# Autodesk Inventor assembly: CCM_Unit
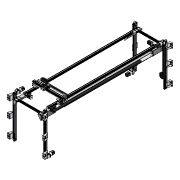
[picture p0: Inventor's stored thumbnail of the model, 180x180]
Saved by Autodesk Inventor 2020 (Build 240168000, 168)
## iProperties
Created: 2021-02-24
Part Number: CCM_Unit
Document SubType Name: Assembly
Designer: magnarecta
Author: magnarecta
## Documents named in this file (19)
- D:\Documents\GitHub\Eto_Project\Hardware\Asem\CCM_Unit.iam
- D:\Documents\GitHub\Eto_Project\Hardware\Parts\CCM\CCM motion linear guide rail\CCM_UNIT\CCM_Unit_C.iam
- D:\Documents\GitHub\Eto_Project\Hardware\Parts\CCM\CCM motion linear guide rail\CCM_UNIT\CCM_Unit_B.iam
- D:\Documents\GitHub\Eto_Project\Hardware\Parts\Stepper_Motor\NEMA23 Stepper.ipt
- D:\Documents\GitHub\Eto_Project\Hardware\Parts\CCM\CCM motion linear guide rail\CCM_UNIT\CCM_Unit_D.iam
- D:\Documents\GitHub\Eto_Project\Hardware\Parts\Meviy\New_Meviy\CCM_Mount_B.ipt
- D:\Documents\GitHub\Eto_Project\Hardware\Parts\Meviy\New_Meviy\CCM_Mount_C.ipt
- D:\Documents\GitHub\Eto_Project\Hardware\Parts\Meviy\New_Meviy\CCM_Mount_D.ipt
- D:\Documents\GitHub\Eto_Project\Hardware\Parts\Meviy\New_Meviy\CCM_Mount_E.ipt
- D:\Documents\GitHub\Eto_Project\Hardware\Parts\Meviy\New_Meviy\CCM_Mount_F.ipt
- D:\Documents\GitHub\Eto_Project\Hardware\Parts\Meviy\New_Meviy\CCM_Mount_G.ipt
- D:\Documents\GitHub\Eto_Project\Hardware\Parts\MISUMI\SLHSSW10_Autodesk_Inventor_2020_20211206\AIS2020\SLHSSW10.iam
- D:\Documents\GitHub\Eto_Project\Hardware\Parts\MISUMI\PSSFGW10-582-M6-N6_Autodesk_Inventor_2020_20211206\PSSFGW10-582-M6-N6.ipt
- D:\Documents\GitHub\Eto_Project\Hardware\Parts\Cable chain\J15BF.1.30_Xaxis.ipt
- D:\Documents\GitHub\Eto_Project\Hardware\Parts\Cable chain\J15BF.1.30_Yaxis.ipt
- D:\Documents\GitHub\Eto_Project\Hardware\Parts\Meviy\New_Meviy\DragChain_Guide_A.ipt
- D:\Documents\GitHub\Eto_Project\Hardware\Parts\Cable chain\J15BF.1.30_Zaxis.ipt
- D:\Documents\GitHub\Eto_Project\Hardware\Parts\Meviy\New_Meviy\DragChain_Guide_B.ipt
- D:\Documents\GitHub\Eto_Project\Hardware\Parts\MISUMI\HFSB6-3030-586-HPW_Autodesk_Inventor_2020_20211208\HFSB6-3030-586-HPW.ipt
## Components (40 placed, 18 different names)
1. CCM_Unit_B:1 [sub-assembly] — 挿入:9, 角度:3, メイト:4, メイト:5, 角度:8, メイト:14, メイト:16, フラッシュ:21, 挿入:37, 挿入:38, メイト:36, フラッシュ:23, メイト:41
2. NEMA23 Stepper:1 — 挿入:12, 角度:5
3. NEMA23 Stepper:2 — 挿入:9, 角度:3
4. CCM_Unit_C:2 [sub-assembly] — メイト:8, メイト:9, フラッシュ:13, フラッシュ:14, フラッシュ:15, フラッシュ:18, 挿入:19, 挿入:20
5. CCM_Unit_D:1 [sub-assembly] — 挿入:12, 角度:5, フラッシュ:20, メイト:35, メイト:36, フラッシュ:26
6. CCM_Unit_B:2 [sub-assembly] — メイト:4, メイト:5, 角度:7, フラッシュ:20, 挿入:35, 挿入:36, フラッシュ:21, フラッシュ:22
7. NEMA23 Stepper:4
8. CCM_Unit_C:3 [sub-assembly] — 角度:7, メイト:8, メイト:9, フラッシュ:16, メイト:12, フラッシュ:17, 挿入:17, 挿入:18
9. CCM_Unit_C:4 [sub-assembly] — フラッシュ:16, メイト:12, メイト:13, メイト:14, フラッシュ:17, フラッシュ:19, 挿入:33, 挿入:34
10. CCM_Unit_C:5 [sub-assembly] — フラッシュ:13, 角度:8, フラッシュ:14, フラッシュ:15, メイト:13, フラッシュ:18, フラッシュ:19, メイト:15, 挿入:15, 挿入:16, メイト:45, 挿入:41, 挿入:42
11. CCM_Mount_B:2 — メイト:15, メイト:16, メイト:17, メイト:18, メイト:19, メイト:20, メイト:21, メイト:22, メイト:23, メイト:24, 挿入:15, 挿入:16, メイト:25, フラッシュ:23, メイト:44, 角度:11
12. CCM_Mount_C:1 — メイト:17, メイト:18, メイト:19
13. CCM_Mount_D:1 — メイト:23, メイト:24, メイト:25
14. CCM_Mount_D:2 — メイト:20, メイト:21, メイト:22, メイト:43, 角度:10
15. CCM_Mount_B:3 — 挿入:17, 挿入:18, 挿入:43
16. CCM_Mount_C:2
17. CCM_Mount_D:3
18. CCM_Mount_D:4
19. CCM_Mount_E:1 — 挿入:19, 挿入:20, 挿入:21, 挿入:22, 挿入:23, 挿入:24, 挿入:25, 挿入:26, フラッシュ:22, 挿入:44
20. CCM_Mount_C:3 — 挿入:21, 挿入:22
21. CCM_Mount_D:5 — 挿入:23, 挿入:24
22. CCM_Mount_C:4 — 挿入:25, 挿入:26
23. CCM_Mount_E:2 — 挿入:33, 挿入:34, フラッシュ:30, 角度:12
24. CCM_Mount_C:5
25. CCM_Mount_D:6
26. CCM_Mount_C:6
27. CCM_Mount_F:1 — 挿入:35, 挿入:36, メイト:35, メイト:38, フラッシュ:28
28. CCM_Mount_G:1 — 挿入:37, 挿入:38, メイト:37, 挿入:39, 挿入:40, フラッシュ:27, メイト:39, メイト:40, 角度:9, フラッシュ:29
29. SLHSSW10:1 [sub-assembly] — メイト:37, フラッシュ:24, フラッシュ:25
30. SLHSSW10:2 [sub-assembly] — メイト:38, フラッシュ:24, フラッシュ:25, フラッシュ:26
31. PSSFGW10-582-M6-N6:1 — 挿入:39
32. PSSFGW10-582-M6-N6:2 — 挿入:40
33. J15BF.1.30_Xaxis:2 — フラッシュ:27, フラッシュ:28, メイト:39
34. J15BF.1.30_Yaxis:1 — メイト:40, 角度:9, フラッシュ:29
35. DragChain_Guide_A:1 — メイト:41, フラッシュ:30, フラッシュ:31, フラッシュ:32, メイト:42
36. DragChain_Guide_A:2 — フラッシュ:31, フラッシュ:32, メイト:42, メイト:43
37. J15BF.1.30_Zaxis:1 — メイト:44, 角度:10, メイト:45, フラッシュ:33
38. DragChain_Guide_B:1 — 挿入:41, 挿入:42, フラッシュ:33
39. HFSB6-3030-586-HPW:1 — 挿入:43, 角度:12
40. HFSB6-3030-586-HPW:2 — 挿入:44, 角度:11
## Relationships (103: Mate 40, Insert 33, Flush 21, Angle 9)
- 挿入:9 [Insert] (2 mm): CCM_Unit_B:1 ↔ NEMA23 Stepper:2
- 角度:3 [Angle] (0 deg): CCM_Unit_B:1 ↔ NEMA23 Stepper:2
- 挿入:12 [Insert] (5 mm): NEMA23 Stepper:1 ↔ CCM_Unit_D:1
- 角度:5 [Angle] (0 deg): NEMA23 Stepper:1 ↔ CCM_Unit_D:1
- [Insert] (2 mm): CCM_Unit_B:2 ↔ NEMA23 Stepper:4
- [Angle] (0 deg): CCM_Unit_B:2 ↔ NEMA23 Stepper:4
- メイト:4 [Mate]: CCM_Unit_B:1 ↔ CCM_Unit_B:2
- メイト:5 [Mate]: CCM_Unit_B:1 ↔ CCM_Unit_B:2
- 角度:7 [Angle] (180 deg): CCM_Unit_B:2 ↔ CCM_Unit_C:3
- メイト:8 [Mate]: CCM_Unit_C:2 ↔ CCM_Unit_C:3
- メイト:9 [Mate]: CCM_Unit_C:2 ↔ CCM_Unit_C:3
- [Mate]: CCM_Unit_C:4 ↔ CCM_Unit_C:5
- [Mate]: CCM_Unit_C:4 ↔ CCM_Unit_C:5
- フラッシュ:13 [Flush]: CCM_Unit_C:2 ↔ CCM_Unit_C:5
- 角度:8 [Angle] (180 deg): CCM_Unit_B:1 ↔ CCM_Unit_C:5
- フラッシュ:14 [Flush]: CCM_Unit_C:2 ↔ CCM_Unit_C:5
- フラッシュ:15 [Flush]: CCM_Unit_C:2 ↔ CCM_Unit_C:5
- フラッシュ:16 [Flush]: CCM_Unit_C:3 ↔ CCM_Unit_C:4
- メイト:12 [Mate] (686 mm): CCM_Unit_C:3 ↔ CCM_Unit_C:4
- メイト:13 [Mate] (2488 mm): CCM_Unit_C:4 ↔ CCM_Unit_C:5
- メイト:14 [Mate] (136.5 mm): CCM_Unit_B:1 ↔ CCM_Unit_C:4
- フラッシュ:17 [Flush]: CCM_Unit_C:3 ↔ CCM_Unit_C:4
- フラッシュ:18 [Flush]: CCM_Unit_C:2 ↔ CCM_Unit_C:5
- フラッシュ:19 [Flush]: CCM_Unit_C:4 ↔ CCM_Unit_C:5
- メイト:15 [Mate]: CCM_Unit_C:5 ↔ CCM_Mount_B:2
- メイト:16 [Mate]: CCM_Unit_B:1 ↔ CCM_Mount_B:2
- メイト:17 [Mate]: CCM_Mount_B:2 ↔ CCM_Mount_C:1
- メイト:18 [Mate]: CCM_Mount_B:2 ↔ CCM_Mount_C:1
- メイト:19 [Mate]: CCM_Mount_B:2 ↔ CCM_Mount_C:1
- メイト:20 [Mate]: CCM_Mount_B:2 ↔ CCM_Mount_D:2
- メイト:21 [Mate]: CCM_Mount_B:2 ↔ CCM_Mount_D:2
- メイト:22 [Mate]: CCM_Mount_B:2 ↔ CCM_Mount_D:2
- メイト:23 [Mate]: CCM_Mount_B:2 ↔ CCM_Mount_D:1
- メイト:24 [Mate]: CCM_Mount_B:2 ↔ CCM_Mount_D:1
- 挿入:15 [Insert]: CCM_Unit_C:5 ↔ CCM_Mount_B:2
- 挿入:16 [Insert]: CCM_Unit_C:5 ↔ CCM_Mount_B:2
- メイト:25 [Mate]: CCM_Mount_B:2 ↔ CCM_Mount_D:1
- [Mate]: CCM_Mount_B:3 ↔ CCM_Mount_C:2
- [Mate]: CCM_Mount_B:3 ↔ CCM_Mount_C:2
- [Mate]: CCM_Mount_B:3 ↔ CCM_Mount_C:2
- [Mate]: CCM_Mount_B:3 ↔ CCM_Mount_D:4
- [Mate]: CCM_Mount_B:3 ↔ CCM_Mount_D:4
- [Mate]: CCM_Mount_B:3 ↔ CCM_Mount_D:4
- [Mate]: CCM_Mount_B:3 ↔ CCM_Mount_D:3
- [Mate]: CCM_Mount_B:3 ↔ CCM_Mount_D:3
- [Mate]: CCM_Mount_B:3 ↔ CCM_Mount_D:3
- 挿入:17 [Insert]: CCM_Unit_C:3 ↔ CCM_Mount_B:3
- 挿入:18 [Insert]: CCM_Unit_C:3 ↔ CCM_Mount_B:3
- 挿入:19 [Insert]: CCM_Unit_C:2 ↔ CCM_Mount_E:1
- 挿入:20 [Insert]: CCM_Unit_C:2 ↔ CCM_Mount_E:1
- 挿入:21 [Insert]: CCM_Mount_E:1 ↔ CCM_Mount_C:3
- 挿入:22 [Insert]: CCM_Mount_E:1 ↔ CCM_Mount_C:3
- 挿入:23 [Insert]: CCM_Mount_E:1 ↔ CCM_Mount_D:5
- 挿入:24 [Insert]: CCM_Mount_E:1 ↔ CCM_Mount_D:5
- 挿入:25 [Insert]: CCM_Mount_E:1 ↔ CCM_Mount_C:4
- 挿入:26 [Insert]: CCM_Mount_E:1 ↔ CCM_Mount_C:4
- [Insert]: CCM_Mount_E:2 ↔ CCM_Mount_C:5
- [Insert]: CCM_Mount_E:2 ↔ CCM_Mount_C:5
- [Insert]: CCM_Mount_E:2 ↔ CCM_Mount_D:6
- [Insert]: CCM_Mount_E:2 ↔ CCM_Mount_D:6
- [Insert]: CCM_Mount_E:2 ↔ CCM_Mount_C:6
- [Insert]: CCM_Mount_E:2 ↔ CCM_Mount_C:6
- 挿入:33 [Insert]: CCM_Unit_C:4 ↔ CCM_Mount_E:2
- 挿入:34 [Insert]: CCM_Unit_C:4 ↔ CCM_Mount_E:2
- フラッシュ:20 [Flush] (-27 mm): CCM_Unit_D:1 ↔ CCM_Unit_B:2
- 挿入:35 [Insert]: CCM_Unit_B:2 ↔ CCM_Mount_F:1
- 挿入:36 [Insert]: CCM_Unit_B:2 ↔ CCM_Mount_F:1
- メイト:35 [Mate]: CCM_Unit_D:1 ↔ CCM_Mount_F:1
- フラッシュ:21 [Flush]: CCM_Unit_B:1 ↔ CCM_Unit_B:2
- 挿入:37 [Insert]: CCM_Unit_B:1 ↔ CCM_Mount_G:1
- 挿入:38 [Insert]: CCM_Unit_B:1 ↔ CCM_Mount_G:1
- メイト:36 [Mate] (20 mm): CCM_Unit_B:1 ↔ CCM_Unit_D:1
- フラッシュ:22 [Flush]: CCM_Unit_B:2 ↔ CCM_Mount_E:1
- フラッシュ:23 [Flush]: CCM_Unit_B:1 ↔ CCM_Mount_B:2
- メイト:37 [Mate]: CCM_Mount_G:1 ↔ SLHSSW10:1
- メイト:38 [Mate]: CCM_Mount_F:1 ↔ SLHSSW10:2
- フラッシュ:24 [Flush]: SLHSSW10:1 ↔ SLHSSW10:2
- フラッシュ:25 [Flush]: SLHSSW10:1 ↔ SLHSSW10:2
- フラッシュ:26 [Flush] (5 mm): CCM_Unit_D:1 ↔ SLHSSW10:2
- 挿入:39 [Insert]: CCM_Mount_G:1 ↔ PSSFGW10-582-M6-N6:1
- 挿入:40 [Insert]: CCM_Mount_G:1 ↔ PSSFGW10-582-M6-N6:2
- フラッシュ:27 [Flush]: CCM_Mount_G:1 ↔ J15BF.1.30_Xaxis:2
- フラッシュ:28 [Flush]: CCM_Mount_F:1 ↔ J15BF.1.30_Xaxis:2
- メイト:39 [Mate]: CCM_Mount_G:1 ↔ J15BF.1.30_Xaxis:2
- メイト:40 [Mate]: CCM_Mount_G:1 ↔ J15BF.1.30_Yaxis:1
- 角度:9 [Angle] (0 deg): CCM_Mount_G:1 ↔ J15BF.1.30_Yaxis:1
- フラッシュ:29 [Flush]: CCM_Mount_G:1 ↔ J15BF.1.30_Yaxis:1
- メイト:41 [Mate]: CCM_Unit_B:1 ↔ DragChain_Guide_A:1
- フラッシュ:30 [Flush] (-23.5 mm): CCM_Mount_E:2 ↔ DragChain_Guide_A:1
- フラッシュ:31 [Flush]: DragChain_Guide_A:1 ↔ DragChain_Guide_A:2
- フラッシュ:32 [Flush]: DragChain_Guide_A:1 ↔ DragChain_Guide_A:2
- メイト:42 [Mate]: DragChain_Guide_A:1 ↔ DragChain_Guide_A:2
- メイト:43 [Mate] (10 mm): CCM_Mount_D:2 ↔ DragChain_Guide_A:2
- メイト:44 [Mate]: CCM_Mount_B:2 ↔ J15BF.1.30_Zaxis:1
- 角度:10 [Angle] (180 deg): CCM_Mount_D:2 ↔ J15BF.1.30_Zaxis:1
- メイト:45 [Mate] (20 mm): CCM_Unit_C:5 ↔ J15BF.1.30_Zaxis:1
- 挿入:41 [Insert]: CCM_Unit_C:5 ↔ DragChain_Guide_B:1
- 挿入:42 [Insert]: CCM_Unit_C:5 ↔ DragChain_Guide_B:1
- フラッシュ:33 [Flush]: J15BF.1.30_Zaxis:1 ↔ DragChain_Guide_B:1
- 挿入:43 [Insert]: CCM_Mount_B:3 ↔ HFSB6-3030-586-HPW:1
- 挿入:44 [Insert]: CCM_Mount_E:1 ↔ HFSB6-3030-586-HPW:2
- 角度:11 [Angle] (0 deg): CCM_Mount_B:2 ↔ HFSB6-3030-586-HPW:2
- 角度:12 [Angle] (0 deg): CCM_Mount_E:2 ↔ HFSB6-3030-586-HPW:1
## Named parameters: d53_d35 = 2 mm, d54_d36 = 0 deg, d65_d63 = 0 mm, d66_d64 = 0 mm, d97_d89 = 0 mm, d98_d90 = 0 mm, d99_d91 = 0 mm, d100_d92 = 0 mm, d101_d93 = 0 mm, d102_d96 = 0 mm, d103_d84 = 0 mm, d104_d85 = 0 mm, d105_d86 = 0 mm, d116_d115 = 0 mm, d117_d110 = 0 mm, d118_d111 = 0 mm, d119_d112 = 0 mm, d120_d113 = 0 mm, d121_d114 = 0 mm
